# Autodesk Inventor assembly: Shaft Collar Hex Threaded_MIR
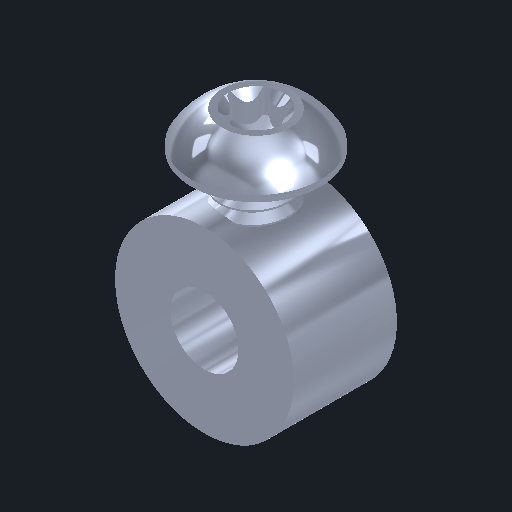
[picture p0: Inventor's stored thumbnail of the model, 512x512]
Saved by Autodesk Inventor 2024 (Build 280153000, 153)
## iProperties
Created: 2022-08-01
Part Number: Shaft Collar Hex Threaded_MIR
Document SubType Name: Assembly
Designer: macbook
Author: ylu12
## Documents named in this file (4)
- \\Mac\Home\Desktop\code\1599V-VRC\Cad\Motion\Shaft LS\Shaft Collar Metal\Shaft Collar Hex Threaded_MIR.iam
- \\Mac\Home\Desktop\code\1599V-VRC\Cad\Motion\Reference Files\Shaft Collar Metal_MIR8.ipt
- \\Mac\Home\Desktop\code\1599V-VRC\Cad\Structure\Hardware\Screw Steel - Star\SScrew Star Threaded .250.ipt
- \\Mac\Home\Desktop\code\1599V-VRC\Cad\Structure\Hardware\Screw Steel - Star.ipt
## Components (2 placed, 2 different names)
1. Shaft Collar Metal_MIR8:1 — Flush:1, Mate:2, Mate:1, Insert:2
2. SScrew Star Threaded .250:1 — Insert:2
## Relationships (4: Mate 2, Flush 1, Insert 1)
- Flush:1: Shaft Collar Metal_MIR8:1
- Mate:2: Shaft Collar Metal_MIR8:1
- Mate:1: Shaft Collar Metal_MIR8:1
- Insert:2 (2.54 mm): Shaft Collar Metal_MIR8:1 ↔ SScrew Star Threaded .250:1
